# Autodesk Inventor assembly: 2x20ExtraTallHeader
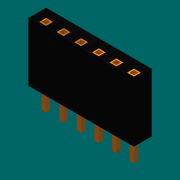
[picture p0: Inventor's stored thumbnail of the model, 180x180]
Saved by Autodesk Inventor 2016 SP1 (Build 200210100, 210)
## iProperties
Created: 2016-04-06
Part Number: 2x20ExtraTallHeader
Document SubType Name: Assembly
Designer: sawai
Author: sawai
## Documents named in this file (2)
- C:\Users\sawai\OneDrive\projects\mppcInterface\cad\connector\2.54Header\female\1x6Female.iam
- C:\Users\sawai\OneDrive\projects\mppcInterface\cad\connector\2.54Header\female\1x1female.iam
## Components (6 placed, 1 different names)
1. 1x1female:1 [sub-assembly]
2. 1x1female:2 [sub-assembly]
3. 1x1female:3 [sub-assembly]
4. 1x1female:4 [sub-assembly]
5. 1x1female:5 [sub-assembly]
6. 1x1female:6 [sub-assembly]
## Component patterns: (6 elements, first: 1x1female:1)
